# Autodesk Inventor assembly: 3dacregconv
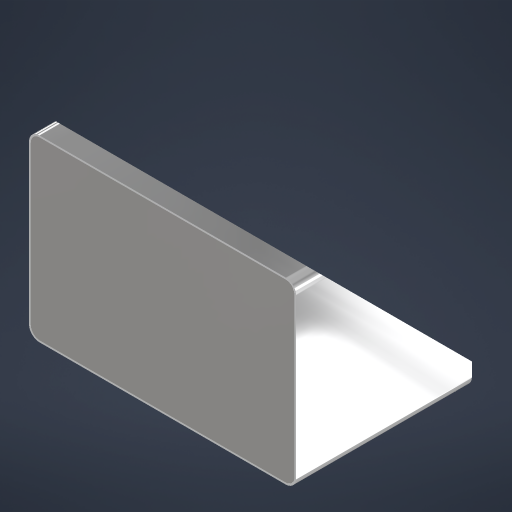
[picture p0: Inventor's stored thumbnail of the model, 512x512]
Saved by Autodesk Inventor 2023 (Build 270158000, 158)
## iProperties
Created: 2022-08-18
Part Number: 3dacregconv
Document SubType Name: Assembly
Designer: HiPeng
Author: HiPeng
## Documents named in this file (4)
- C:\Users\ASUS\Documents\Skripsi\3_phase_firing\3d-cad\3dacregconv.iam
- C:\Users\ASUS\Documents\Skripsi\3_phase_firing\3d-cad\Bottom Cover.ipt
- C:\Users\ASUS\Documents\Skripsi\3_phase_firing\3d-cad\Body Cover.ipt
- C:\Users\ASUS\Documents\Skripsi\3_phase_firing\3d-cad\Top Cover.ipt
## Components (3 placed, 3 different names)
1. Bottom Cover:1 — Flush:1
2. Body Cover:1 — Flush:1, Mate:1, Mate:2, Mate:3, Mate:4
3. Top Cover:1 — Flush:2, Mate:3, Mate:4
## Relationships (6: Mate 4, Flush 2)
- Flush:1: Bottom Cover:1 ↔ Body Cover:1
- Mate:1: Body Cover:1
- Mate:2: Body Cover:1
- Flush:2: Top Cover:1
- Mate:3: Body Cover:1 ↔ Top Cover:1
- Mate:4: Body Cover:1 ↔ Top Cover:1
